# Autodesk Inventor assembly: G81 with Pins
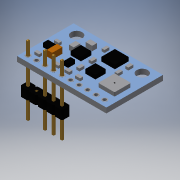
[picture p0: Inventor's stored thumbnail of the model, 180x180]
Saved by Autodesk Inventor 2016 (Build 200138000, 138)
## iProperties
Created: 2015-11-30
Part Number: G81 with Pins
Document SubType Name: Assembly
Designer: Spooner
Author: Spooner
## Documents named in this file (3)
- C:\Users\Spooner\Documents\GY81 Logger\3D Models\G81 with Pins.iam
- C:\Users\Spooner\Documents\GY81 Logger\3D Models\4 Long Male Headers with Gap.ipt
- C:\Users\Spooner\Documents\GY81 Logger\3D Models\GY81.ipt
## Components (2 placed, 2 different names)
1. 4 Long Male Headers with Gap:1 — Mate:1, Mate:2, Mate:3
2. GY81:1 — Mate:1, Mate:2, Mate:3
## Relationships (3: Mate 3)
- Mate:1 (6.35 mm): 4 Long Male Headers with Gap:1 ↔ GY81:1
- Mate:2: 4 Long Male Headers with Gap:1 ↔ GY81:1
- Mate:3: 4 Long Male Headers with Gap:1 ↔ GY81:1
